# Autodesk Inventor assembly: Subsystem_3
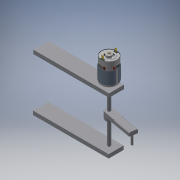
[picture p0: Inventor's stored thumbnail of the model, 180x180]
Saved by Autodesk Inventor 2019.4 (Build 234330000, 330)
## iProperties
Created: 2020-04-15
Part Number: Subsystem_3
Document SubType Name: Assembly
Designer: Niran
Author: Niran
## iProperties of the stored document s.Strikrt.ipt
Created: 2020-04-14
Part Number: s.Strikrt
Material: Generic
Document SubType Name: Modeling
Designer: Darugar
Density: 1 g/cm^3
Appearance: Default
Author: Darugar
Sending System: Autodesk Inventor 2020
## Documents named in this file (6)
- **C:\Users\Niran\Desktop\S.Carrom_bot\Subsystem_3.iam*LocalDocs*xC4yw0hu3Zfgkuz40N05nbvad4b*s.Strikrt.ipt
- C:\Users\Niran\Desktop\S.Carrom_bot\Subsystem_3.iam
- C:\Users\Niran\Desktop\sketch_jan26a\Canon parts\Part36.ipt
- C:\Users\Niran\Desktop\S.Carrom_bot\Part14.ipt
- C:\Users\Niran\Desktop\S.Carrom_bot\DC Motor.ipt
- C:\Users\Niran\Desktop\S.Carrom_bot\s.Strikrt.ipt
## Components (6 placed, 4 different names)
1. Part36:1 — Rotational:3, Rigid:1
2. Part36:2 — Rotational:1, Rotational:2, Rigid:2
3. Part14:1 — Rotational:3
4. Part14:2 — Rotational:1
5. s.Strikrt:1 — Rotational:2, Rigid:1
6. DC Motor:1 — Rigid:2
## Relationships (5: RevoluteJoint 3, WeldJoint 2)
- Rotational:1 [RevoluteJoint]: Part36:2 ↔ Part14:2
- Rotational:2 [RevoluteJoint]: Part36:2 ↔ s.Strikrt:1
- Rotational:3 [RevoluteJoint]: Part36:1 ↔ Part14:1
- Rigid:1 [WeldJoint]: Part36:1 ↔ s.Strikrt:1
- Rigid:2 [WeldJoint] (10 mm): Part36:2 ↔ DC Motor:1
